# Autodesk Inventor assembly: Propeller Motor Guard Assembly
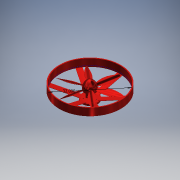
[picture p0: Inventor's stored thumbnail of the model, 180x180]
Saved by Autodesk Inventor 2019 (Build 230136000, 136)
## iProperties
Created: 2020-01-10
Part Number: Propeller Motor Guard Assembly
Document SubType Name: Assembly
Designer: 18186
Author: 18186
## Documents named in this file (4)
- D:\Bike\Propeller Motor Guard Assembly CCW.iam
- D:\Bike\Propeller Guard.ipt
- D:\Bike\12V DC Motor.ipt
- D:\Bike\6 Blade Propeller CCW.ipt
## Components (3 placed, 3 different names)
1. Propeller Guard:1 — Mate:2, Flush:1, Flush:2
2. 12V DC Motor:1 — Mate:2, Flush:1, Flush:2, Mate:3, Mate:4
3. 6 Blade Propeller CCW:1 — Mate:3, Mate:4
## Relationships (5: Mate 3, Flush 2)
- Mate:2: Propeller Guard:1 ↔ 12V DC Motor:1
- Flush:1: Propeller Guard:1 ↔ 12V DC Motor:1
- Flush:2: Propeller Guard:1 ↔ 12V DC Motor:1
- Mate:3: 12V DC Motor:1 ↔ 6 Blade Propeller CCW:1
- Mate:4: 12V DC Motor:1 ↔ 6 Blade Propeller CCW:1
